# Autodesk Inventor assembly: 145pi_tire
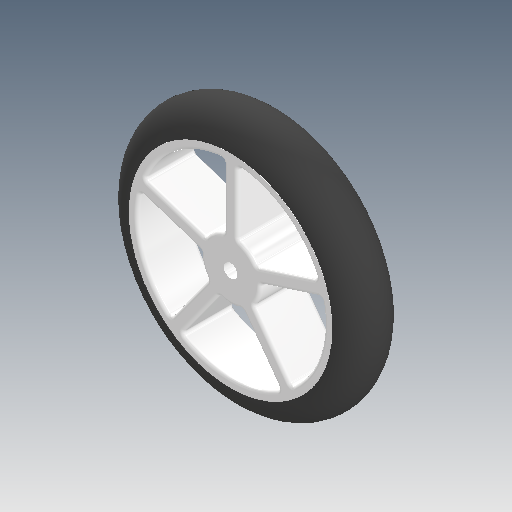
[picture p0: Inventor's stored thumbnail of the model, 512x512]
Saved by Autodesk Inventor 2020 (Build 240168000, 168)
## iProperties
Created: 2020-09-08
Part Number: 145pi_tire
Document SubType Name: Assembly
Designer: 이호석
Mass: 318.31 g
Surface Area: 733.835 cm^2
Volume: 273.774 cm^3
Density: 1.16267 g/cm^3
Author: 이호석
## Documents named in this file (3)
- C:\Inventor\Embedded_contest\145pi_wheel\145pi_tire.iam
- C:\Inventor\Embedded_contest\145pi_wheel\wheel.ipt
- C:\Inventor\Embedded_contest\145pi_wheel\tire.ipt
## Components (2 placed, 2 different names)
1. wheel:1 — 삽입:1, 삽입:2
2. tire:1 — 삽입:1, 삽입:2
## Relationships (2: Insert 2)
- 삽입:1 [Insert]: wheel:1 ↔ tire:1
- 삽입:2 [Insert]: wheel:1 ↔ tire:1
